# Autodesk Inventor assembly: ServoAssemblyActual
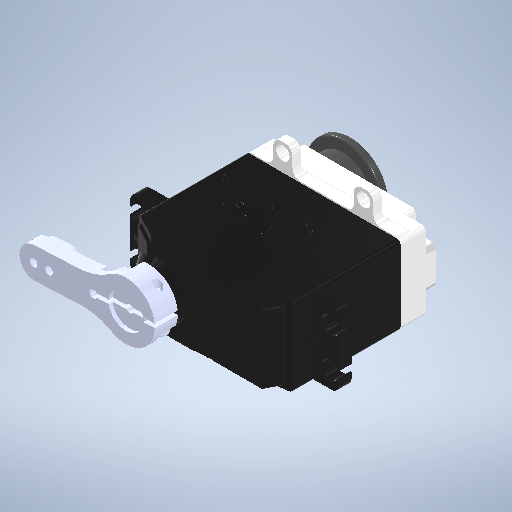
[picture p0: Inventor's stored thumbnail of the model, 512x512]
Saved by Autodesk Inventor 2026.2 (Build 302298010, 298A)
## iProperties
Created: 2026-03-14
Part Number: ServoAssemblyActual
Document SubType Name: Assembly
Designer: Liam
Author: Liam
## Documents named in this file (5)
- C:\Users\Liam\OneDrive\Documents\Inventor\Hexapod\V2\ServoAssemblyActual.iam
- C:\Users\Liam\OneDrive\Documents\Inventor\Hexapod\DS3240NoBottom.ipt
- C:\Users\Liam\OneDrive\Documents\Inventor\Hexapod\V2\ServoCase10mmSideExit.ipt
- C:\Users\Liam\OneDrive\Documents\Inventor\Hexapod\V2\AxleCap.ipt
- C:\Users\Liam\OneDrive\Documents\Inventor\Hexapod\V2\Metal Servo Arm.iam
## Components (4 placed, 4 different names)
1. DS3240NoBottom:1 — Rigid:1, Rigid:3
2. ServoCase10mmSideExit:1 — Rigid:1, Rigid:2
3. AxleCap:1 — Rigid:2
4. Metal Servo Arm:1 [sub-assembly] — Rigid:3
## Relationships (3: WeldJoint 3)
- Rigid:1 [WeldJoint]: DS3240NoBottom:1 ↔ ServoCase10mmSideExit:1
- Rigid:2 [WeldJoint]: ServoCase10mmSideExit:1 ↔ AxleCap:1
- Rigid:3 [WeldJoint]: DS3240NoBottom:1 ↔ Metal Servo Arm:1
